# Autodesk Inventor assembly: chamber_assembly_3Dprint_bee
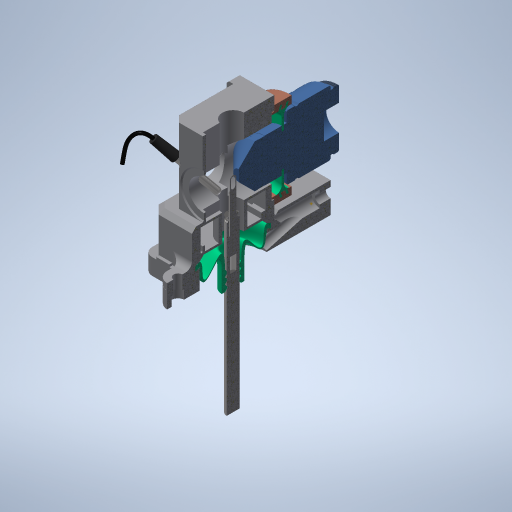
[picture p0: Inventor's stored thumbnail of the model, 512x512]
Saved by Autodesk Inventor 2023.3 (Build 273359000, 359)
## iProperties
Created: 2023-02-16
Part Number: chamber_assembly_3Dprint_bee
Document SubType Name: Assembly
Designer: splath
Author: splath
## Documents named in this file (11)
- Z:\groups\stelzer-opticlab\CAD\mDSLM\New\chamber\chamber_assembly_3Dprint_bee.iam
- Z:\groups\stelzer-opticlab\CAD\mDSLM\New\chamber\objective_sealing\Sealingring_holder.ipt
- Z:\groups\stelzer-opticlab\CAD\mDSLM\New\chamber\bottom_rod_sealing\smooth_bellows\rod_seal_friction.ipt
- Z:\groups\stelzer-opticlab\CAD\mDSLM\New\chamber\objective_sealing\Sealingring.ipt
- Z:\groups\stelzer-opticlab\CAD\DSLM_accessories\specimen_holder\specimen_holder_rod_6mm.ipt
- Z:\groups\stelzer-opticlab\CAD\mDSLM\New\chamber\chamber bottom seal plate.ipt
- Z:\groups\stelzer-opticlab\CAD\mDSLM\New\TempSensor_RS-762-1134.ipt
- Z:\groups\stelzer-opticlab\CAD\mDSLM\New\chamber\bottom_rod_sealing\smooth_bellows\rod_seal_friction_folded.ipt
- Z:\groups\stelzer-opticlab\CAD\mDSLM\New\chamber\zeiss N-Achroplan 10x.ipt
- Z:\groups\stelzer-opticlab\CAD\mDSLM\New\chamber\chamber_V2.2_bee_10x.ipt
- Z:\groups\stelzer-opticlab\CAD\Other\With\Frederic\CopwebHolder_5mm.ipt
## Components (10 placed, 10 different names)
1. chamber_V2.2_bee_10x:1 — Angle:1, Rotational:1
2. chamber bottom seal plate:1
3. Sealingring_holder:1 — Insert:4
4. rod_seal_friction:1 — Mate:2, Rigid:2
5. Sealingring:1 — Insert:4
6. specimen_holder_rod_6mm:1 — Mate:2
7. CopwebHolder_5mm:1 — Angle:1
8. TempSensor_RS-762-1134:1 — Rotational:1
9. rod_seal_friction_folded:1 — Rigid:2
10. zeiss N-Achroplan 10x:1
## Relationships (12: Mate 5, Insert 4, Angle 1, WeldJoint 1, RevoluteJoint 1)
- [Insert]: chamber_V2.2_bee_10x:1 ↔ chamber bottom seal plate:1
- [Mate]: chamber_V2.2_bee_10x:1 ↔ chamber bottom seal plate:1
- [Insert]: chamber_V2.2_bee_10x:1 ↔ Sealingring_holder:1
- [Insert]: chamber_V2.2_bee_10x:1 ↔ rod_seal_friction:1
- Insert:4: Sealingring_holder:1 ↔ Sealingring:1
- Mate:2: rod_seal_friction:1 ↔ specimen_holder_rod_6mm:1
- [Mate]: specimen_holder_rod_6mm:1 ↔ CopwebHolder_5mm:1
- Angle:1 (0 deg): chamber_V2.2_bee_10x:1 ↔ CopwebHolder_5mm:1
- Rigid:2 [WeldJoint]: rod_seal_friction:1 ↔ rod_seal_friction_folded:1
- [Mate]: chamber_V2.2_bee_10x:1 ↔ zeiss N-Achroplan 10x:1
- [Mate] (2.7 mm): chamber_V2.2_bee_10x:1 ↔ zeiss N-Achroplan 10x:1
- Rotational:1 [RevoluteJoint] (4 mm): chamber_V2.2_bee_10x:1 ↔ TempSensor_RS-762-1134:1
## Named parameters: Sealing_offset = 0 mm
